# Autodesk Inventor assembly: Metabox Drawer
Saved by Autodesk Inventor 2024 (Build 280153000, 153)
## iProperties
RuleStatus: InUse
Category: Drawer
AfterAnyParamChange0: Change Skeleton Parameters
AfterComponentSuppressionChange0: Change Skeleton Parameters
AfterComponentReplace0: Change Skeleton Parameters
Created: 2015-04-24
Part Number: Metabox Drawer
Document SubType Name: Assembly
Designer: SauliusD
Description: Metabox Drawer
Author: SauliusD
## Documents named in this file (8)
- C:\W4INV 2024 Design\iBOX LIBRARY\Drawers\Metabox Drawer\Metabox Drawer.iam
- C:\W4INV 2024 Design\iBOX LIBRARY\Drawers\Metabox Drawer\Parts\Metall Box.ipt
- C:\W4INV 2024 Design\iBOX LIBRARY\Drawers\Metabox Drawer\Parts\Fixied Rails.ipt
- C:\W4INV 2024 Design\iBOX LIBRARY\Drawers\Metabox Drawer\Parts\Front Holding Plate.ipt
- C:\W4INV 2024 Design\iBOX LIBRARY\Drawers\Metabox Drawer\Parts\Metabox Bottom.ipt
- C:\W4INV 2024 Design\iBOX LIBRARY\Drawers\Metabox Drawer\Parts\Metabox Back.ipt
- C:\W4INV 2024 Design\iBOX LIBRARY\Drawers\Metabox Drawer\Metalbox Drawer.ipt
- C:\W4INV 2023 Design\iBOX LIBRARY\Drawers\Metalbox Drawer\Metalbox Drawer.iam
## Components (6 placed, 6 different names)
1. @Skeleton — Flush:1, Flush:2, Flush:3, Flush:4, Flush:5, Flush:6, Flush:7, Flush:8, Flush:9, Flush:10, Flush:11, Flush:12, Flush:16, Flush:17, Mate:1
2. Metall Box:1 — Flush:1, Flush:2, Flush:3
3. Fixied Rails:1 — Flush:4, Flush:5, Flush:6
4. Front Holding Plate:1 — Flush:7, Flush:8, Flush:9
5. Metabox Bottom:1 — Flush:10, Flush:11, Flush:12
6. Metabox Back:1 — Flush:16, Flush:17, Mate:1
## Relationships (15: Flush 14, Mate 1)
- Flush:1: @Skeleton ↔ Metall Box:1
- Flush:2: @Skeleton ↔ Metall Box:1
- Flush:3: @Skeleton ↔ Metall Box:1
- Flush:4: @Skeleton ↔ Fixied Rails:1
- Flush:5: @Skeleton ↔ Fixied Rails:1
- Flush:6: @Skeleton ↔ Fixied Rails:1
- Flush:7: @Skeleton ↔ Front Holding Plate:1
- Flush:8: @Skeleton ↔ Front Holding Plate:1
- Flush:9: @Skeleton ↔ Front Holding Plate:1
- Flush:10: @Skeleton ↔ Metabox Bottom:1
- Flush:11: @Skeleton ↔ Metabox Bottom:1
- Flush:12: @Skeleton ↔ Metabox Bottom:1
- Flush:16: @Skeleton ↔ Metabox Back:1
- Flush:17: @Skeleton ↔ Metabox Back:1
- Mate:1: @Skeleton ↔ Metabox Back:1
## Named parameters: Inlet = 0 mm, Board_Thickness = 18 mm, Drawer_Height = 86 mm, Minimal_Back_Space = 10 mm, Distance_from_bottom = 0 mm, Slide_Length = 270 mm
